# Autodesk Inventor assembly: Flywheel Flipper V1
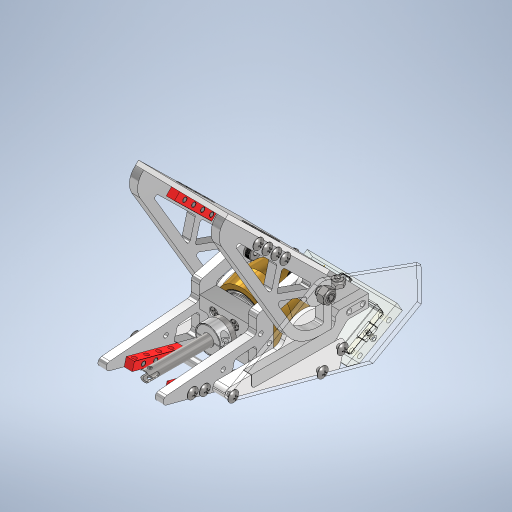
[picture p0: Inventor's stored thumbnail of the model, 512x512]
Saved by Autodesk Inventor 2023.2 (Build 272271000, 271)
## iProperties
Created: 2024-01-10
Part Number: Flywheel Flipper V1
Document SubType Name: Assembly
Designer: Nathan Cai
Mass: 850.1 g
Surface Area: 1945.3 cm^2
Volume: 280.521 cm^3
Density: 3.03043 g/cm^3
Author: Nathan Cai
## Documents named in this file (49)
- E:\Documents\Inventor\Flipper V0.1\Flywheel Flipper V1.iam
- E:\Documents\Inventor\Flipper V0.1\Shaft.ipt
- E:\Documents\Inventor\Flipper V0.1\Bushing.ipt
- E:\Documents\Inventor\Flipper V0.1\Clutch.ipt
- E:\Documents\Inventor\Flipper V0.1\Flywheel.ipt
- E:\Documents\Inventor\Flipper V0.1\98541A119_External Retaining Ring\98541A119_External Retaining Ring.ipt
- E:\Documents\Inventor\Flipper V0.1\98541A420_External Retaining Ring\98541A420_External Retaining Ring.ipt
- E:\Documents\Inventor\Flipper V0.1\Temp - Can.ipt
- E:\Documents\Inventor\Flipper V0.1\Base.ipt
- E:\Documents\Inventor\Flipper V0.1\Temp - Coils.ipt
- E:\Documents\Inventor\Flipper V0.1\Temp - Thrust Bearing.ipt
- E:\Documents\Inventor\Flipper V0.1\Cup.ipt
- E:\Documents\Inventor\Flipper V0.1\Bracket.ipt
- E:\Documents\Inventor\Flipper V0.1\Uprights.ipt
- E:\Documents\Inventor\Flipper V0.1\Arms.ipt
- E:\Documents\Inventor\Flipper V0.1\Rack - Top.ipt
- E:\Documents\Inventor\Flipper V0.1\1561T742_Stacked Wave Disc Spring\1561T742_Stacked Wave Disc Spring.ipt
- E:\Documents\Inventor\Flipper V0.1\4668K148_Permanently Lubricated Stainless Steel Ball Bearing\4668K148_Permanently Lubricated Stainless Steel Ball Bearing.ipt
- E:\Documents\Inventor\Flipper V0.1\9731N46_Clamping Two-Piece Shaft Collar\9731N46_Clamping Two-Piece Shaft Collar.ipt
- E:\Documents\Inventor\Flipper V0.1\Teeth.ipt
- E:\Documents\Inventor\Flipper V0.1\Lever.ipt
- E:\Documents\Inventor\Flipper V0.1\BB 13x19x4.ipt
- E:\Documents\Inventor\Flipper V0.1\1-4in ID Ball Bearing.ipt
- E:\Documents\Inventor\Flipper V0.1\ramp.ipt
- E:\Documents\Inventor\Flipper V0.1\Standoff 1in.ipt
- E:\Documents\Inventor\Flipper V0.1\Uprights - Cover.ipt
- E:\Documents\Inventor\Flipper V0.1\Cam - Shell.ipt
- E:\Documents\Inventor\Flipper V0.1\Cam - Lever.ipt
- E:\Documents\Inventor\Flipper V0.1\Lever - Free.ipt
- E:\Documents\Inventor\Flipper V0.1\8mm x 16mm Flanged Ball Bearing\8mm x 16mm Flanged Ball Bearing.ipt
- E:\Documents\Inventor\Content Center Files\R2023\en-US\ANSI B18.6.3(12)\ANSI B18.6.3 - 6-32 UNC - 0.75(15_).ipt
- E:\Documents\Inventor\Content Center Files\R2023\en-US\ANSI B18.6.3(27)\ANSI B18.6.3 - 6-32 UNC - 0.5(11).ipt
- E:\Documents\Inventor\Content Center Files\R2023\en-US\ANSI B18.6.3(27)\ANSI B18.6.3 - 6-32 UNC - 1(11).ipt
- E:\Documents\Inventor\Flipper V0.1\91259A539_Alloy Steel Shoulder Screw\91259A539_Alloy Steel Shoulder Screw.ipt
- E:\Documents\Inventor\Flipper V0.1\90631A011_Low-Strength Steel Nylon-Insert Locknut\90631A011_Low-Strength Steel Nylon-Insert Locknut.ipt
- E:\Documents\Inventor\Flipper V0.1\Nut Strip 4x4.ipt
- E:\Documents\Inventor\Flipper V0.1\Nut Strip 2x1.ipt
- E:\Documents\Inventor\Flipper V0.1\Exports\Ramp.ipt
- E:\Documents\Inventor\Flipper V0.1\Glider.ipt
- E:\Documents\Inventor\Flipper V0.1\Glider_MIR.ipt
- E:\Documents\Inventor\Flipper V0.1\Exports\Spacer.ipt
- E:\Documents\Inventor\Content Center Files\R2023\en-US\ANSI B18.3(12)\ANSI B18.3 - 6-32 UNC - 0.375(29).ipt
- E:\Documents\Inventor\Flipper V0.1\Exports\Roller.ipt
- E:\Documents\Inventor\Content Center Files\R2023\en-US\ANSI B18.6.3(12)\ANSI B18.6.3 - 6-32 UNC - 0.375(15_).ipt
- E:\Documents\Inventor\Content Center Files\R2023\en-US\SAE J773b\SAE J773b - No. 6. SAE Type L. narrow.ipt
- E:\Documents\Inventor\Content Center Files\R2023\en-US\ANSI B18.2.2(06)\ANSI B18.2.2 - 6 - 32(06).ipt
- E:\Documents\Inventor\Flipper V0.1\Part1\Part1.ipt
- E:\Documents\Inventor\Content Center Files\R2023\en-US\IFI 100 107(2)\IFI 100_107 - No. 6 - 32 Metal Type.ipt
- E:\Documents\Inventor\Flipper V0.1\Exports\Servo Support.ipt
## Components (94 placed, 48 different names)
1. Shaft:1 — Mate:3, Mate:4, Mate:15, Mate:29, Mate:46, Mate:67, Mate:73, Mate:74, Mate:82, Flush:50, Mate:19, Mate:24, Mate:98, Mate:152, Mate:153, Mate:155
2. Bushing:1 — Mate:3, Mate:4, Mate:5, Mate:7, Mate:13, Mate:34, Mate:116, Mate:117
3. Clutch:1 — Mate:5, Mate:7, Mate:14, Mate:34
4. Flywheel:1 — Mate:19, Mate:20, Mate:21, Mate:46, Mate:89, Mate:90, Mate:97, Mate:150, Mate:154
5. 98541A119_External Retaining Ring:1 — Mate:15, Mate:67
6. 98541A420_External Retaining Ring:1 — Mate:13, Mate:14
7. Temp - Can:1 — Mate:20, Mate:21, Mate:22
8. Base:1 — Mate:22, Mate:24, Mate:26, Mate:39, Mate:42, Mate:72, Mate:91, Mate:200
9. Temp - Coils:1 — Mate:26, Mate:200
10. Temp - Thrust Bearing:1 — Mate:29, Mate:40, Mate:99
11. Cup:1 — Mate:75, Tangent:1, Mate:118, Mate:119
12. Bracket:1 — Mate:39, Mate:40, Mate:42, Flush:48, Mate:47, Mate:48, Mate:49, Mate:50, Mate:51, Mate:52, Mate:72, Mate:156, Mate:310, Mate:311, Mate:312, Mate:313
13. Uprights:1 — Mate:47, Mate:48, Mate:49, Mate:70, Mate:71, Mate:115, Mate:137, Mate:139, Angle:1, Mate:180, Mate:181, Mate:195, Mate:196, Flush:63, Mate:241, Mate:242, Mate:243, Mate:245, Mate:240, Mate:306, Mate:307, Mate:308, Mate:309, Angle:2
14. Uprights:2 — Mate:50, Mate:51, Mate:52, Mate:68, Mate:69, Mate:134, Mate:142, Mate:182, Mate:183, Mate:197, Flush:64, Mate:199, Mate:238, Mate:239, Mate:247, Mate:302, Mate:303, Mate:304, Mate:305
15. Uprights - Cover:1 — Mate:133, Mate:134, Mate:185, Mate:283, Mate:284, Mate:285, Mate:286, Mate:287, Mate:288
16. Uprights - Cover:2 — Mate:136, Mate:137, Mate:187, Mate:289, Mate:290, Mate:292, Mate:293, Mate:294
17. Arms:1 — Mate:68, Mate:69, Flush:49, Mate:133, Flush:65, Mate:208, Mate:258, Mate:259, Mate:260, Mate:261, Mate:262, Mate:263, Mate:264, Mate:265
18. Arms:2 — Mate:70, Mate:71, Flush:49, Mate:136, Rotation/Translation:1, Angle:1, Mate:207, Transitional:4, Mate:250, Mate:251, Mate:252, Mate:253, Mate:254, Mate:255, Mate:256, Mate:257
19. Rack - Top:1 — Mate:109, Flush:53, Flush:54, Mate:110, Flush:55, Flush:56, Mate:123, Flush:57, Mate:155, Mate:173, Mate:335, Mate:337
20. ramp:1 — Mate:123, Flush:57, Transitional:3, Mate:173, Mate:332, Mate:333, Mate:334, Mate:336
21. 1561T742_Stacked Wave Disc Spring:1 — Mate:82, Flush:50
22. 4668K148_Permanently Lubricated Stainless Steel Ball Bearing:1 — Mate:89, Mate:90, Mate:91
23. 9731N46_Clamping Two-Piece Shaft Collar:1 — Mate:98, Mate:99
24. Teeth:1 — Mate:109, Flush:53, Flush:54
25. Teeth:2 — Mate:110, Flush:55, Flush:56, Rotation/Translation:1, Flush:66, Mate:244, Transitional:4
26. Lever:1 — Mate:115, Tangent:1, Mate:120, Mate:121, Mate:131, Mate:139, Mate:163, Mate:164, Mate:295, Mate:296, Mate:298, Mate:299, Mate:300, Mate:301
27. Lever - Free:1 — Mate:165, Mate:166
28. BB 13x19x4:1 — Mate:116, Mate:117, Mate:118, Mate:119
29. 1-4in ID Ball Bearing:1 — Mate:120, Mate:121, Transitional:3
30. 1-4in ID Ball Bearing:2 — Mate:130
31. Standoff 1in:1 — Mate:130, Mate:131
32. Standoff 1in:2 — Mate:142
33. Cam - Shell:1 — Mate:145, Mate:146, Mate:315
34. Cam - Lever:1 — Mate:145, Mate:146, Mate:314, Flush:67
35. 8mm x 16mm Flanged Ball Bearing:1 — Mate:150, Mate:153, Mate:154
36. 8mm x 16mm Flanged Ball Bearing:2 — Mate:152, Mate:156
37. 91259A539_Alloy Steel Shoulder Screw:1 — Mate:180, Mate:181, Mate:186, Mate:246
38. 91259A539_Alloy Steel Shoulder Screw:2 — Mate:182, Mate:183, Mate:184, Mate:248
39. 90631A011_Low-Strength Steel Nylon-Insert Locknut:1 — Mate:186, Mate:187
40. 90631A011_Low-Strength Steel Nylon-Insert Locknut:2 — Mate:184, Mate:185
41. Nut Strip 4x4:2
42. Nut Strip 4x4:1
43. Nut Strip 4x4:3 — Mate:195, Mate:210, Mate:274
44. Nut Strip 4x4:4
45. Nut Strip 2x1:1 — Mate:196, Flush:63, Mate:198
46. Nut Strip 2x1:2 — Mate:197, Flush:64, Mate:198, Mate:199
47. Ramp:1 — Mate:207, Flush:65, Mate:208, Mate:266, Mate:267, Mate:268, Mate:269, Mate:270, Mate:271, Mate:272, Mate:273
48. Standoff 1in:3 — Mate:210, Mate:274
49. Glider:1 — Mate:238, Mate:239, Mate:240
50. Glider_MIR:1 — Mate:241, Mate:242, Mate:243, Flush:66, Mate:244, Mate:291
51. Spacer:1 — Mate:245, Mate:246
52. Spacer:2 — Mate:247, Mate:248
53. Roller:1 — Mate:295, Mate:296, Flush:67
54. Part1:1 — Mate:314, Mate:315, Angle:2, Mate:328, Mate:330, Mate:331
55. Servo Support:1 — Mate:328, Mate:330, Mate:331
56. Cross Recessed Flat Countersunk Head Machine Screw - Type I - Inch 6-32 x 3/4:5 — Mate:332
57. Prevailing Torque Type Hex Nut - Inch (IFI) No. 6 - 32 Metal Type:2 — Mate:336, Mate:337
58. Cross Recessed Flat Countersunk Head Machine Screw - Type I - Inch 6-32 x 3/4:6 — Mate:333
59. Prevailing Torque Type Hex Nut - Inch (IFI) No. 6 - 32 Metal Type:1 — Mate:334, Mate:335
60. Cross Recessed Truss Head Machine Screw - Type I - Inch No. 6 - 32 - 1/2:3 — Mate:250, Mate:251
61. Cross Recessed Truss Head Machine Screw - Type I - Inch No. 6 - 32 - 1/2:4 — Mate:252, Mate:253
62. Cross Recessed Truss Head Machine Screw - Type I - Inch No. 6 - 32 - 1/2:5 — Mate:254, Mate:255
63. Cross Recessed Truss Head Machine Screw - Type I - Inch No. 6 - 32 - 1/2:6 — Mate:256, Mate:257
64. Cross Recessed Truss Head Machine Screw - Type I - Inch No. 6 - 32 - 1/2:7 — Mate:258, Mate:259
65. Cross Recessed Truss Head Machine Screw - Type I - Inch No. 6 - 32 - 1/2:8 — Mate:260, Mate:261
66. Cross Recessed Truss Head Machine Screw - Type I - Inch No. 6 - 32 - 1/2:9 — Mate:262, Mate:263
67. Cross Recessed Truss Head Machine Screw - Type I - Inch No. 6 - 32 - 1/2:10 — Mate:264, Mate:265
68. Spline Socket Flat Countersunk Head Cap Screw - Inch 6-32 UNC x 0.375:1 — Mate:266
69. Spline Socket Flat Countersunk Head Cap Screw - Inch 6-32 UNC x 0.375:2 — Mate:267
70. Spline Socket Flat Countersunk Head Cap Screw - Inch 6-32 UNC x 0.375:3 — Mate:268
71. Spline Socket Flat Countersunk Head Cap Screw - Inch 6-32 UNC x 0.375:4 — Mate:269
72. Spline Socket Flat Countersunk Head Cap Screw - Inch 6-32 UNC x 0.375:5 — Mate:270
73. Spline Socket Flat Countersunk Head Cap Screw - Inch 6-32 UNC x 0.375:6 — Mate:271
74. Spline Socket Flat Countersunk Head Cap Screw - Inch 6-32 UNC x 0.375:7 — Mate:272
75. Spline Socket Flat Countersunk Head Cap Screw - Inch 6-32 UNC x 0.375:8 — Mate:273
76. Cross Recessed Truss Head Machine Screw - Type I - Inch No. 6 - 32 - 1:5 — Mate:285, Mate:286
77. Cross Recessed Truss Head Machine Screw - Type I - Inch No. 6 - 32 - 1:6 — Mate:287, Mate:288
78. Cross Recessed Truss Head Machine Screw - Type I - Inch No. 6 - 32 - 1:7 — Mate:291, Mate:292
79. Cross Recessed Truss Head Machine Screw - Type I - Inch No. 6 - 32 - 1:8 — Mate:293, Mate:294
80. Cross Recessed Flat Countersunk Head Machine Screw - Type I - Inch 6-32 x 3/8:1 — Mate:300, Mate:301
81. Conical Spring Washer SAE J773b (Inch) No. 6. SAE Type L. narrow:1 — Mate:298, Mate:299, Insert:1
82. Hex Machine Screw Nut - Inch 6 - 32:1 — Insert:1
83. Cross Recessed Truss Head Machine Screw - Type I - Inch No. 6 - 32 - 1/2:11 — Mate:302, Mate:303
84. Cross Recessed Truss Head Machine Screw - Type I - Inch No. 6 - 32 - 1/2:12 — Mate:304, Mate:305
85. Cross Recessed Truss Head Machine Screw - Type I - Inch No. 6 - 32 - 1/2:13 — Mate:306, Mate:307
86. Cross Recessed Truss Head Machine Screw - Type I - Inch No. 6 - 32 - 1/2:14 — Mate:308, Mate:309
87. Cross Recessed Flat Countersunk Head Machine Screw - Type I - Inch 6-32 x 3/4:1 — Mate:310
88. Cross Recessed Flat Countersunk Head Machine Screw - Type I - Inch 6-32 x 3/4:2 — Mate:311
89. Cross Recessed Flat Countersunk Head Machine Screw - Type I - Inch 6-32 x 3/4:3 — Mate:312
90. Cross Recessed Flat Countersunk Head Machine Screw - Type I - Inch 6-32 x 3/4:4 — Mate:313
91. Cross Recessed Truss Head Machine Screw - Type I - Inch No. 6 - 32 - 1:1 — Mate:289, Mate:290
92. Cross Recessed Truss Head Machine Screw - Type I - Inch No. 6 - 32 - 1:2 — Mate:283, Mate:284
93. Cross Recessed Truss Head Machine Screw - Type I - Inch No. 6 - 32 - 1/2:1 — Mate:163, Mate:164
94. Cross Recessed Truss Head Machine Screw - Type I - Inch No. 6 - 32 - 1/2:2 — Mate:165, Mate:166
## Relationships (203: Mate 179, Flush 17, Transitional 2, Angle 2, Tangent 1, RelateRotateTranslate 1, Insert 1)
- Mate:3: Shaft:1 ↔ Bushing:1
- Mate:4: Shaft:1 ↔ Bushing:1
- Mate:5: Bushing:1 ↔ Clutch:1
- Mate:7: Bushing:1 ↔ Clutch:1
- Mate:13: Bushing:1 ↔ 98541A420_External Retaining Ring:1
- Mate:14: Clutch:1 ↔ 98541A420_External Retaining Ring:1
- Mate:15: Shaft:1 ↔ 98541A119_External Retaining Ring:1
- Mate:19: Shaft:1 ↔ Flywheel:1
- Mate:20: Flywheel:1 ↔ Temp - Can:1
- Mate:21: Flywheel:1 ↔ Temp - Can:1
- Mate:22: Temp - Can:1 ↔ Base:1
- Mate:24: Shaft:1 ↔ Base:1
- Mate:26: Base:1 ↔ Temp - Coils:1
- Mate:29: Shaft:1 ↔ Temp - Thrust Bearing:1
- Mate:34: Bushing:1 ↔ Clutch:1
- Mate:39: Base:1 ↔ Bracket:1
- Mate:40: Temp - Thrust Bearing:1 ↔ Bracket:1
- Mate:42: Base:1 ↔ Bracket:1
- Mate:46: Shaft:1 ↔ Flywheel:1
- Flush:48: Bracket:1
- Mate:47: Bracket:1 ↔ Uprights:1
- Mate:48: Bracket:1 ↔ Uprights:1
- Mate:49: Bracket:1 ↔ Uprights:1
- Mate:50: Bracket:1 ↔ Uprights:2
- Mate:51: Bracket:1 ↔ Uprights:2
- Mate:52: Bracket:1 ↔ Uprights:2
- Mate:67: Shaft:1 ↔ 98541A119_External Retaining Ring:1
- Mate:68 (3.175 mm): Uprights:2 ↔ Arms:1
- Mate:69: Uprights:2 ↔ Arms:1
- Mate:70 (3.175 mm): Uprights:1 ↔ Arms:2
- Mate:71: Uprights:1 ↔ Arms:2
- Flush:49: Arms:1 ↔ Arms:2
- Mate:72: Base:1 ↔ Bracket:1
- Mate:73: Shaft:1
- Mate:74: Shaft:1
- Mate:75: Cup:1
- Mate:82: Shaft:1 ↔ 1561T742_Stacked Wave Disc Spring:1
- Flush:50: Shaft:1 ↔ 1561T742_Stacked Wave Disc Spring:1
- Mate:89: Flywheel:1 ↔ 4668K148_Permanently Lubricated Stainless Steel Ball Bearing:1
- Mate:90: Flywheel:1 ↔ 4668K148_Permanently Lubricated Stainless Steel Ball Bearing:1
- Mate:91: Base:1 ↔ 4668K148_Permanently Lubricated Stainless Steel Ball Bearing:1
- Mate:97: Flywheel:1
- Mate:98: Shaft:1 ↔ 9731N46_Clamping Two-Piece Shaft Collar:1
- Mate:99: Temp - Thrust Bearing:1 ↔ 9731N46_Clamping Two-Piece Shaft Collar:1
- Mate:109: Rack - Top:1 ↔ Teeth:1
- Flush:53: Rack - Top:1 ↔ Teeth:1
- Flush:54: Rack - Top:1 ↔ Teeth:1
- Mate:110: Rack - Top:1 ↔ Teeth:2
- Flush:55: Rack - Top:1 ↔ Teeth:2
- Flush:56: Rack - Top:1 ↔ Teeth:2
- Mate:115: Uprights:1 ↔ Lever:1
- Tangent:1: Cup:1 ↔ Lever:1
- Mate:116: Bushing:1 ↔ BB 13x19x4:1
- Mate:117: Bushing:1 ↔ BB 13x19x4:1
- Mate:118: Cup:1 ↔ BB 13x19x4:1
- Mate:119: Cup:1 ↔ BB 13x19x4:1
- Mate:120: Lever:1 ↔ 1-4in ID Ball Bearing:1
- Mate:121 (1 mm): Lever:1 ↔ 1-4in ID Ball Bearing:1
- Mate:123: Rack - Top:1 ↔ ramp:1
- Flush:57: Rack - Top:1 ↔ ramp:1
- [Mate]: Uprights:2 ↔ Lever - Free:1
- [Mate]: Lever:1 ↔ Lever - Free:1
- [Mate] (1 mm): Lever - Free:1 ↔ 1-4in ID Ball Bearing:2
- [Mate]: Lever - Free:1 ↔ 1-4in ID Ball Bearing:2
- Mate:130: 1-4in ID Ball Bearing:2 ↔ Standoff 1in:1
- Mate:131: Lever:1 ↔ Standoff 1in:1
- Mate:133: Uprights - Cover:1 ↔ Arms:1
- Mate:134: Uprights:2 ↔ Uprights - Cover:1
- Mate:136: Uprights - Cover:2 ↔ Arms:2
- Mate:137: Uprights:1 ↔ Uprights - Cover:2
- Mate:139: Uprights:1 ↔ Lever:1
- Transitional:3: ramp:1 ↔ 1-4in ID Ball Bearing:1
- [Mate]: Uprights:2 ↔ Lever - Free:1
- [Mate]: Lever - Free:1 ↔ Standoff 1in:2
- Mate:142: Uprights:2 ↔ Standoff 1in:2
- Mate:145: Cam - Shell:1 ↔ Cam - Lever:1
- Mate:146: Cam - Shell:1 ↔ Cam - Lever:1
- Mate:150: Flywheel:1 ↔ 8mm x 16mm Flanged Ball Bearing:1
- Mate:152: Shaft:1 ↔ 8mm x 16mm Flanged Ball Bearing:2
- Mate:153: Shaft:1 ↔ 8mm x 16mm Flanged Ball Bearing:1
- Mate:154: Flywheel:1 ↔ 8mm x 16mm Flanged Ball Bearing:1
- Rotation/Translation:1 [RelateRotateTranslate] (149.6187 mm): Arms:2 ↔ Teeth:2
- Mate:155 (3.175 mm): Shaft:1 ↔ Rack - Top:1
- Angle:1 (60 deg): Uprights:1 ↔ Arms:2
- Mate:156: Bracket:1 ↔ 8mm x 16mm Flanged Ball Bearing:2
- Mate:163: Lever:1 ↔ Cross Recessed Truss Head Machine Screw - Type I - Inch No. 6 - 32 - 1/2:1
- Mate:164: Lever:1 ↔ Cross Recessed Truss Head Machine Screw - Type I - Inch No. 6 - 32 - 1/2:1
- Mate:165: Lever - Free:1 ↔ Cross Recessed Truss Head Machine Screw - Type I - Inch No. 6 - 32 - 1/2:2
- Mate:166: Lever - Free:1 ↔ Cross Recessed Truss Head Machine Screw - Type I - Inch No. 6 - 32 - 1/2:2
- Mate:173: Rack - Top:1 ↔ ramp:1
- Mate:180: Uprights:1 ↔ 91259A539_Alloy Steel Shoulder Screw:1
- Mate:181: Uprights:1 ↔ 91259A539_Alloy Steel Shoulder Screw:1
- Mate:182: Uprights:2 ↔ 91259A539_Alloy Steel Shoulder Screw:2
- Mate:183: Uprights:2 ↔ 91259A539_Alloy Steel Shoulder Screw:2
- Mate:184: 91259A539_Alloy Steel Shoulder Screw:2 ↔ 90631A011_Low-Strength Steel Nylon-Insert Locknut:2
- Mate:185: Uprights - Cover:1 ↔ 90631A011_Low-Strength Steel Nylon-Insert Locknut:2
- Mate:186: 91259A539_Alloy Steel Shoulder Screw:1 ↔ 90631A011_Low-Strength Steel Nylon-Insert Locknut:1
- Mate:187: Uprights - Cover:2 ↔ 90631A011_Low-Strength Steel Nylon-Insert Locknut:1
- [Mate]: Arms:2 ↔ Nut Strip 4x4:2
- [Flush]: Arms:2 ↔ Nut Strip 4x4:2
- [Mate]: Arms:2 ↔ Nut Strip 4x4:2
- [Mate]: Arms:1 ↔ Nut Strip 4x4:1
- [Mate]: Arms:1 ↔ Nut Strip 4x4:1
- [Mate]: Arms:1 ↔ Nut Strip 4x4:1
- [Flush]: Uprights:1 ↔ Nut Strip 4x4:3
- [Mate]: Uprights:1 ↔ Nut Strip 4x4:3
- [Mate]: Uprights:2 ↔ Nut Strip 4x4:4
- [Flush]: Uprights:2 ↔ Nut Strip 4x4:4
- [Flush]: Nut Strip 4x4:3 ↔ Nut Strip 4x4:4
- Mate:195: Uprights:1 ↔ Nut Strip 4x4:3
- Mate:196: Uprights:1 ↔ Nut Strip 2x1:1
- Flush:63: Uprights:1 ↔ Nut Strip 2x1:1
- Mate:197: Uprights:2 ↔ Nut Strip 2x1:2
- Flush:64: Uprights:2 ↔ Nut Strip 2x1:2
- Mate:198: Nut Strip 2x1:1 ↔ Nut Strip 2x1:2
- Mate:199: Uprights:2 ↔ Nut Strip 2x1:2
- Mate:200: Base:1 ↔ Temp - Coils:1
- Mate:207: Arms:2 ↔ Ramp:1
- Flush:65: Arms:1 ↔ Ramp:1
- Mate:208: Arms:1 ↔ Ramp:1
- Mate:210: Nut Strip 4x4:3 ↔ Standoff 1in:3
- Mate:238: Uprights:2 ↔ Glider:1
- Mate:239: Uprights:2 ↔ Glider:1
- Mate:240: Uprights:1 ↔ Glider:1
- Mate:241: Uprights:1 ↔ Glider_MIR:1
- Mate:242: Uprights:1 ↔ Glider_MIR:1
- Mate:243: Uprights:1 ↔ Glider_MIR:1
- Flush:66: Teeth:2 ↔ Glider_MIR:1
- Mate:244: Teeth:2 ↔ Glider_MIR:1
- Mate:245: Uprights:1 ↔ Spacer:1
- Mate:246: 91259A539_Alloy Steel Shoulder Screw:1 ↔ Spacer:1
- Mate:247: Uprights:2 ↔ Spacer:2
- Mate:248: 91259A539_Alloy Steel Shoulder Screw:2 ↔ Spacer:2
- Transitional:4: Arms:2 ↔ Teeth:2
- Mate:250: Arms:2 ↔ Cross Recessed Truss Head Machine Screw - Type I - Inch No. 6 - 32 - 1/2:3
- Mate:251: Arms:2 ↔ Cross Recessed Truss Head Machine Screw - Type I - Inch No. 6 - 32 - 1/2:3
- Mate:252: Arms:2 ↔ Cross Recessed Truss Head Machine Screw - Type I - Inch No. 6 - 32 - 1/2:4
- Mate:253: Arms:2 ↔ Cross Recessed Truss Head Machine Screw - Type I - Inch No. 6 - 32 - 1/2:4
- Mate:254: Arms:2 ↔ Cross Recessed Truss Head Machine Screw - Type I - Inch No. 6 - 32 - 1/2:5
- Mate:255: Arms:2 ↔ Cross Recessed Truss Head Machine Screw - Type I - Inch No. 6 - 32 - 1/2:5
- Mate:256: Arms:2 ↔ Cross Recessed Truss Head Machine Screw - Type I - Inch No. 6 - 32 - 1/2:6
- Mate:257: Arms:2 ↔ Cross Recessed Truss Head Machine Screw - Type I - Inch No. 6 - 32 - 1/2:6
- Mate:258: Arms:1 ↔ Cross Recessed Truss Head Machine Screw - Type I - Inch No. 6 - 32 - 1/2:7
- Mate:259: Arms:1 ↔ Cross Recessed Truss Head Machine Screw - Type I - Inch No. 6 - 32 - 1/2:7
- Mate:260: Arms:1 ↔ Cross Recessed Truss Head Machine Screw - Type I - Inch No. 6 - 32 - 1/2:8
- Mate:261: Arms:1 ↔ Cross Recessed Truss Head Machine Screw - Type I - Inch No. 6 - 32 - 1/2:8
- Mate:262: Arms:1 ↔ Cross Recessed Truss Head Machine Screw - Type I - Inch No. 6 - 32 - 1/2:9
- Mate:263: Arms:1 ↔ Cross Recessed Truss Head Machine Screw - Type I - Inch No. 6 - 32 - 1/2:9
- Mate:264: Arms:1 ↔ Cross Recessed Truss Head Machine Screw - Type I - Inch No. 6 - 32 - 1/2:10
- Mate:265: Arms:1 ↔ Cross Recessed Truss Head Machine Screw - Type I - Inch No. 6 - 32 - 1/2:10
- Mate:266: Ramp:1 ↔ Spline Socket Flat Countersunk Head Cap Screw - Inch 6-32 UNC x 0.375:1
- Mate:267: Ramp:1 ↔ Spline Socket Flat Countersunk Head Cap Screw - Inch 6-32 UNC x 0.375:2
- Mate:268: Ramp:1 ↔ Spline Socket Flat Countersunk Head Cap Screw - Inch 6-32 UNC x 0.375:3
- Mate:269: Ramp:1 ↔ Spline Socket Flat Countersunk Head Cap Screw - Inch 6-32 UNC x 0.375:4
- Mate:270: Ramp:1 ↔ Spline Socket Flat Countersunk Head Cap Screw - Inch 6-32 UNC x 0.375:5
- Mate:271: Ramp:1 ↔ Spline Socket Flat Countersunk Head Cap Screw - Inch 6-32 UNC x 0.375:6
- Mate:272: Ramp:1 ↔ Spline Socket Flat Countersunk Head Cap Screw - Inch 6-32 UNC x 0.375:7
- Mate:273: Ramp:1 ↔ Spline Socket Flat Countersunk Head Cap Screw - Inch 6-32 UNC x 0.375:8
- Mate:274: Nut Strip 4x4:3 ↔ Standoff 1in:3
- Mate:283: Uprights - Cover:1 ↔ Cross Recessed Truss Head Machine Screw - Type I - Inch No. 6 - 32 - 1:2
- Mate:284: Uprights - Cover:1 ↔ Cross Recessed Truss Head Machine Screw - Type I - Inch No. 6 - 32 - 1:2
- Mate:285: Uprights - Cover:1 ↔ Cross Recessed Truss Head Machine Screw - Type I - Inch No. 6 - 32 - 1:5
- Mate:286: Uprights - Cover:1 ↔ Cross Recessed Truss Head Machine Screw - Type I - Inch No. 6 - 32 - 1:5
- Mate:287: Uprights - Cover:1 ↔ Cross Recessed Truss Head Machine Screw - Type I - Inch No. 6 - 32 - 1:6
- Mate:288: Uprights - Cover:1 ↔ Cross Recessed Truss Head Machine Screw - Type I - Inch No. 6 - 32 - 1:6
- Mate:289: Uprights - Cover:2 ↔ Cross Recessed Truss Head Machine Screw - Type I - Inch No. 6 - 32 - 1:1
- Mate:290: Uprights - Cover:2 ↔ Cross Recessed Truss Head Machine Screw - Type I - Inch No. 6 - 32 - 1:1
- Mate:291: Glider_MIR:1 ↔ Cross Recessed Truss Head Machine Screw - Type I - Inch No. 6 - 32 - 1:7
- Mate:292: Uprights - Cover:2 ↔ Cross Recessed Truss Head Machine Screw - Type I - Inch No. 6 - 32 - 1:7
- Mate:293: Uprights - Cover:2 ↔ Cross Recessed Truss Head Machine Screw - Type I - Inch No. 6 - 32 - 1:8
- Mate:294: Uprights - Cover:2 ↔ Cross Recessed Truss Head Machine Screw - Type I - Inch No. 6 - 32 - 1:8
- Mate:295: Lever:1 ↔ Roller:1
- Mate:296: Lever:1 ↔ Roller:1
- Mate:298: Lever:1 ↔ Conical Spring Washer SAE J773b (Inch) No. 6. SAE Type L. narrow:1
- Mate:299: Lever:1 ↔ Conical Spring Washer SAE J773b (Inch) No. 6. SAE Type L. narrow:1
- Insert:1: Conical Spring Washer SAE J773b (Inch) No. 6. SAE Type L. narrow:1 ↔ Hex Machine Screw Nut - Inch 6 - 32:1
- Mate:300: Lever:1 ↔ Cross Recessed Flat Countersunk Head Machine Screw - Type I - Inch 6-32 x 3/8:1
- Mate:301: Lever:1 ↔ Cross Recessed Flat Countersunk Head Machine Screw - Type I - Inch 6-32 x 3/8:1
- Mate:302: Uprights:2 ↔ Cross Recessed Truss Head Machine Screw - Type I - Inch No. 6 - 32 - 1/2:11
- Mate:303: Uprights:2 ↔ Cross Recessed Truss Head Machine Screw - Type I - Inch No. 6 - 32 - 1/2:11
- Mate:304: Uprights:2 ↔ Cross Recessed Truss Head Machine Screw - Type I - Inch No. 6 - 32 - 1/2:12
- Mate:305: Uprights:2 ↔ Cross Recessed Truss Head Machine Screw - Type I - Inch No. 6 - 32 - 1/2:12
- Mate:306: Uprights:1 ↔ Cross Recessed Truss Head Machine Screw - Type I - Inch No. 6 - 32 - 1/2:13
- Mate:307: Uprights:1 ↔ Cross Recessed Truss Head Machine Screw - Type I - Inch No. 6 - 32 - 1/2:13
- Mate:308: Uprights:1 ↔ Cross Recessed Truss Head Machine Screw - Type I - Inch No. 6 - 32 - 1/2:14
- Mate:309: Uprights:1 ↔ Cross Recessed Truss Head Machine Screw - Type I - Inch No. 6 - 32 - 1/2:14
- Mate:310: Bracket:1 ↔ Cross Recessed Flat Countersunk Head Machine Screw - Type I - Inch 6-32 x 3/4:1
- Mate:311: Bracket:1 ↔ Cross Recessed Flat Countersunk Head Machine Screw - Type I - Inch 6-32 x 3/4:2
- Mate:312: Bracket:1 ↔ Cross Recessed Flat Countersunk Head Machine Screw - Type I - Inch 6-32 x 3/4:3
- Mate:313: Bracket:1 ↔ Cross Recessed Flat Countersunk Head Machine Screw - Type I - Inch 6-32 x 3/4:4
- Mate:314: Cam - Lever:1 ↔ Part1:1
- Mate:315: Cam - Shell:1 ↔ Part1:1
- Angle:2 (45 deg): Uprights:1 ↔ Part1:1
- Flush:67: Cam - Lever:1 ↔ Roller:1
- Mate:328: Part1:1 ↔ Servo Support:1
- Mate:330: Part1:1 ↔ Servo Support:1
- Mate:331: Part1:1 ↔ Servo Support:1
- Mate:332: ramp:1 ↔ Cross Recessed Flat Countersunk Head Machine Screw - Type I - Inch 6-32 x 3/4:5
- Mate:333: ramp:1 ↔ Cross Recessed Flat Countersunk Head Machine Screw - Type I - Inch 6-32 x 3/4:6
- Mate:334: ramp:1 ↔ Prevailing Torque Type Hex Nut - Inch (IFI) No. 6 - 32 Metal Type:1
- Mate:335: Rack - Top:1 ↔ Prevailing Torque Type Hex Nut - Inch (IFI) No. 6 - 32 Metal Type:1
- Mate:336: ramp:1 ↔ Prevailing Torque Type Hex Nut - Inch (IFI) No. 6 - 32 Metal Type:2
- Mate:337: Rack - Top:1 ↔ Prevailing Torque Type Hex Nut - Inch (IFI) No. 6 - 32 Metal Type:2
